# Autodesk Inventor assembly: Feeder
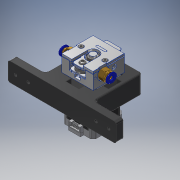
[picture p0: Inventor's stored thumbnail of the model, 180x180]
Saved by Autodesk Inventor 2017 (Build 210142000, 142)
## iProperties
Company: FABLAB Frenchmakers
Part Number: Feeder
Material: Générique
Document SubType Name: Assembly
Designer: FABLAB Frenchmakers
Project: 1420 Vauban 3D XL
Catalog Web Link: http://frenchmakers.com/
Stock Number: 1420-05-10
## Documents named in this file (3)
- W:\Professionnel\Conception FABLAB\1420-Vauban 3D XL\1420-05 Feeder\1420-05-10 Feeder.iam
- W:\Professionnel\Conception FABLAB\1420-Vauban 3D XL\1420-05 Feeder\1420-05-01 Support moteur.ipt
- W:\Professionnel\Conception FABLAB\1420-Vauban 3D XL\1420-05 Feeder\1420-05-10 Bulldog feeder.iam
## Components (2 placed, 2 different names)
1. 1420-05-01 Support moteur:1 — Placage:1, Placage:2, Placage:3
2. 1420-05-10 Bulldog feeder:1 [sub-assembly] — Placage:1, Placage:2, Placage:3
## Relationships (3: Mate 3)
- Placage:1 [Mate]: 1420-05-01 Support moteur:1 ↔ 1420-05-10 Bulldog feeder:1
- Placage:2 [Mate]: 1420-05-01 Support moteur:1 ↔ 1420-05-10 Bulldog feeder:1
- Placage:3 [Mate]: 1420-05-01 Support moteur:1 ↔ 1420-05-10 Bulldog feeder:1
